# Autodesk Inventor assembly: Robot Assembly - 6 wheel - toughbox mini - 26x28 official version
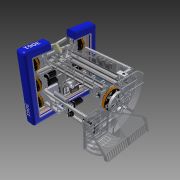
[picture p0: Inventor's stored thumbnail of the model, 180x180]
Saved by Autodesk Inventor 2013 (Build 170138000, 138)
## iProperties
Created: 2013-01-06
Part Number: Robot Assembly - 6 wheel - toughbox mini - 26x28 official version
Document SubType Name: Assembly
Designer: Moses
Mass: 49932.1 g
Surface Area: 138154 cm^2
Volume: 42618.2 cm^3
Density: 1.17161 g/cm^3
Author: Moses
## Documents named in this file (66)
- C:\Users\Arpan\Documents\GitHub\frc2013CAD\Robot Assembly - 6 wheel - toughbox mini - 26x28 official version.iam
- C:\Users\Arpan\Documents\GitHub\frc2013CAD\Drivetrain\Bearings\fr8zz-hex.ipt
- C:\Users\Arpan\Documents\GitHub\frc2013CAD\Drivetrain\Drive Wheel Assembly V2.iam
- C:\Users\Arpan\Documents\GitHub\frc2013CAD\Drivetrain\Standard Wheel Assembly V2.iam
- C:\Users\Arpan\Documents\GitHub\frc2013CAD\Drivetrain\Toughbox-mini\Toughbox-mini-hex-long.iam
- C:\Users\Arpan\Documents\GitHub\frc2013CAD\Drivetrain\6157K140 Shaft Collar\6157K140.ipt
- C:\Users\Arpan\Documents\GitHub\frc2013CAD\Drivetrain\Shaft Spacer Part1.ipt
- C:\Users\Arpan\Documents\GitHub\frc2013CAD\Drivetrain\Shaft Spacer Part2.ipt
- C:\Users\Arpan\Documents\GitHub\frc2013CAD\Drivetrain\Shaft Spacer Part3.ipt
- C:\Users\Arpan\Documents\GitHub\frc2013CAD\Drivetrain\Shaft Spacer Part4.ipt
- C:\Users\Arpan\Documents\GitHub\frc2013CAD\Drivetrain\Shaft Spacer Part5.ipt
- C:\Users\Arpan\Documents\GitHub\frc2013CAD\Drivetrain\Shaft Spacer Part6.ipt
- C:\Users\Arpan\Documents\GitHub\frc2013CAD\Drivetrain\6061K130 Shaft\6061K130.ipt
- C:\Users\Arpan\Documents\GitHub\frc2013CAD\Electrical\ELEC_CircuitBreaker_CB185-120.iam
- C:\Users\Arpan\Documents\GitHub\frc2013CAD\Electrical\CS_compactRIO_cRIO-FRC-II.ipt
- C:\Users\Arpan\Documents\GitHub\frc2013CAD\Electrical\CS_WirelessBridge_DAP1522.ipt
- C:\Users\Arpan\Documents\GitHub\frc2013CAD\Drivetrain\Pneumatic_Compressor_VIAIR_00090\Pneumatic_Compressor_VIAIR_00090.iam
- C:\Users\Arpan\Documents\GitHub\frc2013CAD\Drivetrain\Mounting Bracket V1.500 - (toughbox-mini - sheet metal).ipt
- C:\Users\Arpan\Documents\GitHub\frc2013CAD\Drivetrain\Mounting Bracket V1.500 - (toughbox-mini - sheet metal - underside).ipt
- C:\Users\Arpan\Documents\GitHub\frc2013CAD\Drivetrain\Bearing Block V1.500 Drivetrain.ipt
- C:\Users\Arpan\Documents\GitHub\frc2013CAD\Drivetrain\Shaft Mount V1.500 Drivetrain.ipt
- C:\Users\Arpan\Documents\GitHub\frc2013CAD\Launcher\Shooter\Shooter Assembly v2.iam
- C:\Users\Arpan\Documents\GitHub\frc2013CAD\Chassis\Chassis Assembly 26x28 Version\Chassis Assembly 26x28 Version.iam
- C:\Users\Arpan\Documents\GitHub\frc2013CAD\Chassis\Bumpers\Bumper Assembly1 (26x28 robot).iam
- C:\Users\Arpan\Documents\GitHub\frc2013CAD\Climber rough space budget version\arm assembly mount plate.ipt
- C:\Users\Arpan\Documents\GitHub\frc2013CAD\Cimber actual\main climber.iam
- C:\Users\Arpan\Documents\GitHub\frc2013CAD\Electrical\Mounting Board 3.ipt
- C:\Users\Arpan\Documents\GitHub\frc2013CAD\Drivetrain\Wheel Mount Support Plate - drive wheel.ipt
- C:\Users\Arpan\Documents\GitHub\frc2013CAD\Drivetrain\Wheel Mount Support Plate.ipt
- C:\Users\Arpan\Documents\GitHub\frc2013CAD\Chassis\Bumpers\Bumper Assembly2 (26x28 robot).iam
- C:\Users\Arpan\Documents\GitHub\frc2013CAD\Chassis\Bumpers\Bumper Assembly3 (26x28 robot).iam
- C:\Users\Arpan\Documents\GitHub\frc2013CAD\Chassis\Bumpers\Bumper Assembly4 (26x28 robot).iam
- C:\Users\Arpan\Documents\GitHub\frc2013CAD\Electrical\Electrical Board 1.iam
- C:\Users\Arpan\Documents\GitHub\frc2013CAD\Cimber actual\Arm Motor\arm bearing support.iam
- C:\Users\Arpan\Documents\GitHub\frc2013CAD\Cimber actual\Arm Motor\bracket for PG-71.ipt
- C:\Users\Arpan\Documents\GitHub\frc2013CAD\Cimber actual\Arm Motor\Imported Components\5972K322 bearing for motor\5972K322 bearing for motor.ipt
- C:\Users\Arpan\Documents\GitHub\frc2013CAD\Cimber actual\Arm Motor\Imported Components\PG-71-am-0914\PG-71-am-0914.ipt
- C:\Users\Arpan\Documents\GitHub\frc2013CAD\Cimber actual\Winch mount assenbly.iam
- C:\Users\Arpan\Documents\GitHub\frc2013CAD\Cimber actual\bearing 3 8 ths OD.ipt
- C:\Users\Arpan\Documents\GitHub\frc2013CAD\Cimber actual\14 inch shaft.ipt
- C:\Users\Arpan\Documents\GitHub\frc2013CAD\Cimber actual\winch support.ipt
- C:\Users\Arpan\Documents\GitHub\frc2013CAD\Cimber actual\anti - chain tension.ipt
- C:\Users\Arpan\Documents\GitHub\frc2013CAD\Cimber actual\spacer plate.ipt
- C:\Users\Arpan\Documents\GitHub\frc2013CAD\Cimber actual\V mount.ipt
- C:\Users\Arpan\Documents\GitHub\frc2013CAD\Cimber actual\nylon thing.ipt
- C:\Users\Arpan\Documents\GitHub\frc2013CAD\Cimber actual\p80 support post.iam
- C:\Users\Arpan\Documents\GitHub\frc2013CAD\Cimber actual\that thing mount.ipt
- C:\Users\Arpan\Documents\GitHub\frc2013CAD\Cimber actual\Hub for rachet.ipt
- C:\Users\Arpan\Documents\GitHub\frc2013CAD\Cimber actual\Part4.ipt
- C:\Users\Arpan\Documents\GitHub\frc2013CAD\Cimber actual\rachet gear analouge.ipt
- C:\Users\Arpan\Documents\GitHub\frc2013CAD\Cimber actual\cylinder.iam
- C:\Users\Arpan\Documents\GitHub\frc2013CAD\Cimber actual\tiny clevis.ipt
- C:\Users\Arpan\Documents\GitHub\frc2013CAD\Cimber actual\tube v.iam
- C:\Users\Arpan\Documents\GitHub\frc2013CAD\Cimber actual\paul mount.ipt
- C:\Users\Arpan\Documents\GitHub\frc2013CAD\Cimber actual\cylinder mount.ipt
- C:\Users\Arpan\Documents\GitHub\frc2013CAD\Cimber actual\passive hooks arpan style.iam.ipt
- C:\Users\Arpan\Documents\GitHub\frc2013CAD\Cimber actual\winch mount back support.ipt
- C:\Users\Arpan\Documents\GitHub\frc2013CAD\Cimber actual\ninja.ipt
- C:\Users\Arpan\Documents\GitHub\frc2013CAD\Climber rough space budget version\arm assembly mount plate 2.ipt
- C:\Users\Arpan\Documents\GitHub\frc2013CAD\Climber rough space budget version\arm assembly mount plate 3.ipt
- C:\Users\Arpan\Documents\GitHub\frc2013CAD\Cimber actual\P80 Mount Assembly V2.iam
- C:\Users\Arpan\Documents\GitHub\frc2013CAD\Cimber actual\Back Brace Mount V2.ipt
- C:\Users\Arpan\Documents\GitHub\frc2013CAD\Electrical\ELEC_Battery_NP18-12B.iam
- C:\Users\Arpan\Documents\GitHub\frc2013CAD\Pneumatics\Pneumatics_Clippard_AVT-32-16.iam
- C:\Users\Arpan\Documents\GitHub\frc2013CAD\Electrical\Circuit Breaker Mount.ipt
- passive hooks arpan style.iam
## Components (107 placed, 64 different names)
1. Chassis Assembly 26x28 Version:1 [sub-assembly] — Mate:1, Flush:1, Mate:2, Flush:4, Mate:3, Mate:4, Mate:5, Mate:8, Mate:9, Mate:10, Mate:17, Mate:18, Mate:19, Mate:20, Mate:21, Mate:26, Mate:27, Mate:28, Mate:29, Mate:34, Mate:35, Mate:36, Mate:37, Mate:42, Mate:43, Mate:44, Mate:47, Mate:48, Mate:51, Mate:52, Mate:55, Mate:83, Mate:84, Mate:85, Mate:89, Mate:98, Mate:99, Mate:100, Mate:101, Mate:115, Mate:116, Mate:117, Mate:118, Mate:119, Mate:120, Mate:125, Mate:126, Mate:127, Mate:128, Mate:129, Mate:130, Mate:132, Mate:136, Mate:153, Flush:17, Mate:154, Mate:155, Mate:159, Mate:190, Flush:162, Flush:191, Mate:194, Mate:195, Mate:196, Mate:197, Mate:198, Mate:199, Mate:200, Mate:201, Mate:202, Mate:203, Mate:204, Mate:205, Mate:206, Mate:207, Mate:208, Mate:209, Mate:210, Mate:211, Mate:212, Mate:213, Mate:214, Mate:215, Mate:216, Mate:217, Mate:218, Mate:219, Mate:220, Mate:221, Mate:222, Mate:223, Mate:249, Flush:193, Flush:194, Angle:4, Mate:255, Mate:256, Flush:196, Flush:197, Flush:204, Mate:271, Flush:206, Angle:5, Mate:278, Flush:208, Mate:279, Mate:282, Mate:284, Mate:286, Flush:213, Mate:288, Flush:214, Mate:289, Flush:216, Flush:222, Mate:310, Mate:311, Mate:312, Flush:233, Mate:316, Mate:317, Flush:235, Flush:237, Mate:319, Flush:238, Mate:321, Flush:239, Mate:323, Flush:215, Flush:217, Angle:11, Mate:328, Mate:329, Mate:330, Mate:331, Mate:332, Mate:333, Mate:334
2. Bumper Assembly1 (26x28 robot):1 [sub-assembly] — Mate:5, Mate:3, Flush:6, Flush:9, Flush:10
3. Bumper Assembly1 (26x28 robot):2 [sub-assembly] — Mate:1, Flush:1, Flush:3, Flush:2, Flush:7, Flush:8
4. Bumper Assembly2 (26x28 robot):1 [sub-assembly] — Mate:2, Flush:2, Flush:3, Flush:4, Mate:5, Flush:10
5. Bumper Assembly3 (26x28 robot):1 [sub-assembly] — Flush:9, Mate:5, Flush:6
6. Bumper Assembly4 (26x28 robot):1 [sub-assembly] — Mate:4, Flush:7, Flush:8
7. Wheel Mount Support Plate - drive wheel:1 — Mate:194, Mate:195, Mate:196
8. Wheel Mount Support Plate - drive wheel:2 — Mate:197, Mate:198, Mate:199
9. Wheel Mount Support Plate:1 — Mate:200, Mate:201, Mate:202
10. Wheel Mount Support Plate:2 — Mate:203, Mate:204, Mate:205
11. Wheel Mount Support Plate:3 — Mate:206, Mate:207, Mate:208
12. Wheel Mount Support Plate:4 — Mate:209, Mate:210, Mate:211
13. Wheel Mount Support Plate:5 — Mate:212, Mate:213, Mate:214
14. Wheel Mount Support Plate:6 — Mate:215, Mate:216, Mate:217
15. Wheel Mount Support Plate:7 — Mate:218, Mate:219, Mate:220
16. Wheel Mount Support Plate:8 — Mate:221, Mate:222, Mate:223
17. Pneumatic_Compressor_VIAIR_00090:1 [sub-assembly] — Mate:144, Mate:240, Mate:241, Mate:244, Mate:245
18. Shaft Spacer Part1:1 — Insert:111
19. Shaft Spacer Part2:1 — Insert:112
20. Shaft Spacer Part1:3 — Insert:113
21. Shaft Spacer Part2:2 — Insert:114
22. Shaft Spacer Part3:1 — Insert:115
23. Shaft Spacer Part3:2 — Insert:116
24. Shaft Spacer Part4:2 — Insert:117
25. Shaft Spacer Part4:1 — Insert:118
26. Shaft Spacer Part5:1 — Insert:119
27. Shaft Spacer Part5:2 — Insert:120
28. Shaft Spacer Part6:1 — Insert:121
29. Shaft Spacer Part6:2 — Insert:122
30. 6157K140:1 — Insert:107, Insert:113
31. 6157K140:2 — Insert:108, Insert:114
32. 6157K140:3 — Insert:110, Insert:111
33. 6157K140:4 — Insert:109, Insert:112
34. Toughbox-mini-hex-long:2 [sub-assembly] — Mate:131, Mate:132, Mate:133, Mate:134, Mate:135, Insert:118
35. Toughbox-mini-hex-long:1 [sub-assembly] — Mate:136, Mate:137, Mate:138, Mate:139, Mate:140, Insert:117
36. fr8zz-hex:1 — Insert:94, Insert:116
37. Bearing Block V1.500 Drivetrain:1 — Mate:83, Mate:84, Mate:85, Insert:106
38. Bearing Block V1.500 Drivetrain:2 — Mate:98, Mate:99, Mate:100, Insert:94
39. fr8zz-hex:2 — Insert:106, Insert:115
40. Mounting Bracket V1.500 - (toughbox-mini - sheet metal):1 — Mate:115, Mate:116, Mate:117, Mate:137, Mate:138
41. Mounting Bracket V1.500 - (toughbox-mini - sheet metal):2 — Mate:118, Mate:119, Mate:120, Mate:131, Mate:133
42. Mounting Bracket V1.500 - (toughbox-mini - sheet metal - underside):1 — Mate:125, Mate:126, Mate:127
43. Mounting Bracket V1.500 - (toughbox-mini - sheet metal - underside):2 — Mate:128, Mate:129, Mate:130
44. Shaft Mount V1.500 Drivetrain:8 — Mate:34, Mate:35, Mate:51, Insert:121
45. Shaft Mount V1.500 Drivetrain:7 — Mate:28, Mate:29, Mate:48, Insert:110
46. Shaft Mount V1.500 Drivetrain:6 — Mate:42, Mate:43, Mate:47, Insert:122
47. Shaft Mount V1.500 Drivetrain:5 — Mate:36, Mate:37, Mate:44, Insert:107
48. Shaft Mount V1.500 Drivetrain:4 — Mate:26, Mate:27, Mate:55, Insert:7, Insert:109
49. Shaft Mount V1.500 Drivetrain:3 — Mate:20, Mate:21, Mate:52, Insert:5, Insert:119
50. Shaft Mount V1.500 Drivetrain:2 — Mate:17, Mate:18, Mate:19, Insert:2, Insert:108
51. Shaft Mount V1.500 Drivetrain:1 — Mate:8, Mate:9, Mate:10, Insert:1, Insert:120
52. 6061K130:4 — Insert:7, Mate:21
53. 6061K130:3 — Insert:5, Mate:22
54. 6061K130:2 — Insert:2, Mate:19
55. 6061K130:1 — Insert:1, Mate:17
56. Standard Wheel Assembly V2:3 [sub-assembly] — Mate:17, Flush:13, Rotation:1
57. Drive Wheel Assembly V2:1 [sub-assembly] — Mate:89, Flush:13, Flush:15, Mate:139, Mate:140, Rotation:1, Rotation:2, Tangent:3
58. Standard Wheel Assembly V2:1 [sub-assembly] — Mate:19, Flush:15, Rotation:2
59. Standard Wheel Assembly V2:2 [sub-assembly] — Mate:21, Flush:11, Rotation:4
60. Standard Wheel Assembly V2:4 [sub-assembly] — Mate:22, Flush:12, Rotation:3
61. Drive Wheel Assembly V2:2 [sub-assembly] — Mate:101, Flush:11, Flush:12, Mate:134, Mate:135, Rotation:3, Rotation:4
62. Circuit Breaker Mount:1 — Mate:335, Mate:246, Mate:338, Mate:13, Mate:339, Mate:340
63. Pneumatics_Clippard_AVT-32-16:1 [sub-assembly] — Tangent:4, Angle:12, Mate:334, Tangent:5
64. ELEC_Battery_NP18-12B:1 [sub-assembly] — Mate:331, Mate:332, Mate:333
65. Mounting Board 3:1 — Mate:190, Flush:162, Mate:16, Mate:188, Mate:189, Flush:191, Mate:144, Mate:240, Mate:241, Mate:244, Mate:245
66. Electrical Board 1:1 [sub-assembly] — Mate:242, Mate:243, Flush:192
67. CS_WirelessBridge_DAP1522:1 — Flush:152, Mate:164, Flush:224
68. CS_compactRIO_cRIO-FRC-II:1 — Mate:16, Mate:188, Mate:189
69. ELEC_CircuitBreaker_CB185-120:1 [sub-assembly] — Mate:246, Mate:338, Mate:13
70. Shooter Assembly v2:1 [sub-assembly] — Mate:153, Flush:17, Mate:154, Mate:159, Mate:164, Flush:152, Flush:224, Mate:242, Mate:243, Flush:192, Mate:258, Mate:285, Flush:211, Mate:326, Flush:240, Tangent:4, Angle:12, Tangent:5
71. main climber:1 [sub-assembly] — Tangent:2, Mate:282, Mate:308, Mate:309, Mate:318, Mate:320, Mate:322, Angle:11
72. arm bearing support:1 [sub-assembly] — Mate:249, Flush:193, Mate:252, Flush:195
73. bracket for PG-71:1 — Flush:194, Mate:253, Mate:323, Mate:324
74. arm assembly mount plate:2 — Mate:155, Mate:318, Flush:237, Mate:328, Mate:329
75. 5972K322 bearing for motor:1 — Mate:252, Flush:195, Mate:254, Mate:325
76. PG-71-am-0914:1 — Mate:253, Mate:254, Mate:324, Mate:325
77. Back Brace Mount V2:1 — Mate:326, Flush:240, Mate:327, Mate:335, Mate:339, Mate:340
78. Winch mount assenbly:1 [sub-assembly] — Mate:255, Flush:197, Mate:257, Mate:258, Mate:259, Mate:262, Mate:269, Mate:270, Flush:205, Flush:234
79. bearing 3 8 ths OD:1 — Mate:259, Mate:262, Mate:263
80. Winch mount assenbly:2 [sub-assembly] — Mate:256, Flush:196, Mate:257, Mate:260, Mate:261, Flush:207, Mate:300, Flush:227, Mate:301, Mate:302, Mate:304, Mate:305, Mate:314, Mate:315
81. bearing 3 8 ths OD:2 — Mate:260, Mate:261
82. 14 inch shaft:1 — Mate:263, Mate:290, Mate:292
83. winch support:2 — Flush:204, Mate:269, Mate:270, Flush:205, Mate:272, Mate:273, Mate:274
84. winch support:3 — Mate:271, Flush:206, Flush:207
85. anti - chain tension:1 — Mate:272, Mate:273, Mate:274, Mate:276, Mate:277
86. spacer plate:1 — Mate:276, Mate:277
87. V mount:1 — Mate:278, Flush:208, Mate:279, Mate:283, Flush:210, Flush:215, Flush:217, Mate:298, Mate:299
88. nylon thing:1 — Mate:283, Mate:284, Flush:210
89. P80 Mount Assembly V2:1 [sub-assembly] — Mate:285, Flush:211, Mate:287, Mate:327
90. that thing mount:1 — Mate:288, Flush:214, Angle:10
91. that thing mount:2 — Mate:289, Flush:216
92. p80 support post:1 [sub-assembly] — Mate:286, Mate:287, Flush:213, Flush:236
93. Hub for rachet:1 — Mate:290, Mate:293
94. Part4:1
95. rachet gear analouge:1 — Mate:292, Mate:293
96. cylinder:1 [sub-assembly] — Mate:306, Angle:6, Flush:229, Mate:307, Flush:230, Flush:231
97. tube v:1 [sub-assembly] — Mate:298, Mate:299, Flush:222
98. paul mount:1 — Mate:300, Flush:227, Mate:301, Flush:228
99. cylinder mount:2 — Mate:304, Flush:228, Mate:305, Angle:7, Mate:307, Flush:230, Flush:231, Mate:302
100. tiny clevis:1 — Mate:306, Angle:6, Angle:7, Flush:229
101. passive hooks arpan style.iam:1 — Mate:308, Mate:311, Angle:9, Angle:10
102. passive hooks arpan style.iam:2 — Mate:309, Mate:310, Angle:9
103. winch mount back support:1 — Mate:312, Flush:233, Flush:234
104. ninja:1 — Mate:317, Flush:235, Flush:236
105. winch mount back support:2 — Mate:314, Mate:315, Mate:316
106. arm assembly mount plate 2:1 — Mate:319, Flush:238, Mate:320, Mate:330
107. arm assembly mount plate 3:1 — Mate:321, Mate:322, Flush:239
## Relationships (273: Mate 185, Flush 50, Insert 22, Angle 8, RelateRotation 4, Tangent 4)
- Mate:1: Chassis Assembly 26x28 Version:1 ↔ Bumper Assembly1 (26x28 robot):2
- Flush:1: Chassis Assembly 26x28 Version:1 ↔ Bumper Assembly1 (26x28 robot):2
- Mate:2: Chassis Assembly 26x28 Version:1 ↔ Bumper Assembly2 (26x28 robot):1
- Flush:2: Bumper Assembly1 (26x28 robot):2 ↔ Bumper Assembly2 (26x28 robot):1
- Flush:3: Bumper Assembly1 (26x28 robot):2 ↔ Bumper Assembly2 (26x28 robot):1
- Flush:4 (-69.85 mm): Chassis Assembly 26x28 Version:1 ↔ Bumper Assembly2 (26x28 robot):1
- Mate:5: Bumper Assembly1 (26x28 robot):1 ↔ Bumper Assembly2 (26x28 robot):1
- Mate:3: Chassis Assembly 26x28 Version:1 ↔ Bumper Assembly1 (26x28 robot):1
- Flush:6: Bumper Assembly1 (26x28 robot):1 ↔ Bumper Assembly3 (26x28 robot):1
- Mate:4: Chassis Assembly 26x28 Version:1 ↔ Bumper Assembly4 (26x28 robot):1
- Flush:7: Bumper Assembly1 (26x28 robot):2 ↔ Bumper Assembly4 (26x28 robot):1
- Flush:8: Bumper Assembly1 (26x28 robot):2 ↔ Bumper Assembly4 (26x28 robot):1
- Flush:9: Bumper Assembly1 (26x28 robot):1 ↔ Bumper Assembly3 (26x28 robot):1
- Flush:10: Bumper Assembly1 (26x28 robot):1 ↔ Bumper Assembly2 (26x28 robot):1
- Mate:5: Chassis Assembly 26x28 Version:1 ↔ Bumper Assembly3 (26x28 robot):1
- Insert:1 (-6.35 mm): Shaft Mount V1.500 Drivetrain:1 ↔ 6061K130:1
- Insert:2 (-6.35 mm): Shaft Mount V1.500 Drivetrain:2 ↔ 6061K130:2
- Insert:5 (-6.35 mm): Shaft Mount V1.500 Drivetrain:3 ↔ 6061K130:3
- Insert:7 (-6.35 mm): Shaft Mount V1.500 Drivetrain:4 ↔ 6061K130:4
- Mate:8: Chassis Assembly 26x28 Version:1 ↔ Shaft Mount V1.500 Drivetrain:1
- Mate:9: Chassis Assembly 26x28 Version:1 ↔ Shaft Mount V1.500 Drivetrain:1
- Mate:10: Chassis Assembly 26x28 Version:1 ↔ Shaft Mount V1.500 Drivetrain:1
- Mate:17: Chassis Assembly 26x28 Version:1 ↔ Shaft Mount V1.500 Drivetrain:2
- Mate:18: Chassis Assembly 26x28 Version:1 ↔ Shaft Mount V1.500 Drivetrain:2
- Mate:19: Chassis Assembly 26x28 Version:1 ↔ Shaft Mount V1.500 Drivetrain:2
- Mate:20: Chassis Assembly 26x28 Version:1 ↔ Shaft Mount V1.500 Drivetrain:3
- Mate:21: Chassis Assembly 26x28 Version:1 ↔ Shaft Mount V1.500 Drivetrain:3
- Mate:26: Chassis Assembly 26x28 Version:1 ↔ Shaft Mount V1.500 Drivetrain:4
- Mate:27: Chassis Assembly 26x28 Version:1 ↔ Shaft Mount V1.500 Drivetrain:4
- Mate:28: Chassis Assembly 26x28 Version:1 ↔ Shaft Mount V1.500 Drivetrain:7
- Mate:29: Chassis Assembly 26x28 Version:1 ↔ Shaft Mount V1.500 Drivetrain:7
- Mate:34: Chassis Assembly 26x28 Version:1 ↔ Shaft Mount V1.500 Drivetrain:8
- Mate:35: Chassis Assembly 26x28 Version:1 ↔ Shaft Mount V1.500 Drivetrain:8
- Mate:36: Chassis Assembly 26x28 Version:1 ↔ Shaft Mount V1.500 Drivetrain:5
- Mate:37: Chassis Assembly 26x28 Version:1 ↔ Shaft Mount V1.500 Drivetrain:5
- Mate:42: Chassis Assembly 26x28 Version:1 ↔ Shaft Mount V1.500 Drivetrain:6
- Mate:43: Chassis Assembly 26x28 Version:1 ↔ Shaft Mount V1.500 Drivetrain:6
- Mate:44: Chassis Assembly 26x28 Version:1 ↔ Shaft Mount V1.500 Drivetrain:5
- Mate:47: Chassis Assembly 26x28 Version:1 ↔ Shaft Mount V1.500 Drivetrain:6
- Mate:48: Chassis Assembly 26x28 Version:1 ↔ Shaft Mount V1.500 Drivetrain:7
- Mate:51: Chassis Assembly 26x28 Version:1 ↔ Shaft Mount V1.500 Drivetrain:8
- Mate:52: Chassis Assembly 26x28 Version:1 ↔ Shaft Mount V1.500 Drivetrain:3
- Mate:55: Chassis Assembly 26x28 Version:1 ↔ Shaft Mount V1.500 Drivetrain:4
- Mate:17: 6061K130:1 ↔ Standard Wheel Assembly V2:3
- Mate:19: 6061K130:2 ↔ Standard Wheel Assembly V2:1
- Mate:21: 6061K130:4 ↔ Standard Wheel Assembly V2:2
- Mate:22: 6061K130:3 ↔ Standard Wheel Assembly V2:4
- Mate:83: Chassis Assembly 26x28 Version:1 ↔ Bearing Block V1.500 Drivetrain:1
- Mate:84: Chassis Assembly 26x28 Version:1 ↔ Bearing Block V1.500 Drivetrain:1
- Mate:85: Chassis Assembly 26x28 Version:1 ↔ Bearing Block V1.500 Drivetrain:1
- Mate:89 (6.35 mm): Chassis Assembly 26x28 Version:1 ↔ Drive Wheel Assembly V2:1
- Insert:94: fr8zz-hex:1 ↔ Bearing Block V1.500 Drivetrain:2
- Mate:98: Chassis Assembly 26x28 Version:1 ↔ Bearing Block V1.500 Drivetrain:2
- Mate:99: Chassis Assembly 26x28 Version:1 ↔ Bearing Block V1.500 Drivetrain:2
- Mate:100: Chassis Assembly 26x28 Version:1 ↔ Bearing Block V1.500 Drivetrain:2
- Mate:101 (6.35 mm): Chassis Assembly 26x28 Version:1 ↔ Drive Wheel Assembly V2:2
- Insert:106: Bearing Block V1.500 Drivetrain:1 ↔ fr8zz-hex:2
- Mate:115: Chassis Assembly 26x28 Version:1 ↔ Mounting Bracket V1.500 - (toughbox-mini - sheet metal):1
- Mate:116: Chassis Assembly 26x28 Version:1 ↔ Mounting Bracket V1.500 - (toughbox-mini - sheet metal):1
- Mate:117: Chassis Assembly 26x28 Version:1 ↔ Mounting Bracket V1.500 - (toughbox-mini - sheet metal):1
- Mate:118: Chassis Assembly 26x28 Version:1 ↔ Mounting Bracket V1.500 - (toughbox-mini - sheet metal):2
- Mate:119: Chassis Assembly 26x28 Version:1 ↔ Mounting Bracket V1.500 - (toughbox-mini - sheet metal):2
- Mate:120: Chassis Assembly 26x28 Version:1 ↔ Mounting Bracket V1.500 - (toughbox-mini - sheet metal):2
- Flush:11: Standard Wheel Assembly V2:2 ↔ Drive Wheel Assembly V2:2
- Flush:12: Standard Wheel Assembly V2:4 ↔ Drive Wheel Assembly V2:2
- Flush:13: Standard Wheel Assembly V2:3 ↔ Drive Wheel Assembly V2:1
- Mate:125: Chassis Assembly 26x28 Version:1 ↔ Mounting Bracket V1.500 - (toughbox-mini - sheet metal - underside):1
- Mate:126: Chassis Assembly 26x28 Version:1 ↔ Mounting Bracket V1.500 - (toughbox-mini - sheet metal - underside):1
- Mate:127: Chassis Assembly 26x28 Version:1 ↔ Mounting Bracket V1.500 - (toughbox-mini - sheet metal - underside):1
- Mate:128: Chassis Assembly 26x28 Version:1 ↔ Mounting Bracket V1.500 - (toughbox-mini - sheet metal - underside):2
- Mate:129: Chassis Assembly 26x28 Version:1 ↔ Mounting Bracket V1.500 - (toughbox-mini - sheet metal - underside):2
- Mate:130: Chassis Assembly 26x28 Version:1 ↔ Mounting Bracket V1.500 - (toughbox-mini - sheet metal - underside):2
- Flush:15: Drive Wheel Assembly V2:1 ↔ Standard Wheel Assembly V2:1
- Mate:131: Toughbox-mini-hex-long:2 ↔ Mounting Bracket V1.500 - (toughbox-mini - sheet metal):2
- Mate:132: Chassis Assembly 26x28 Version:1 ↔ Toughbox-mini-hex-long:2
- Mate:133: Toughbox-mini-hex-long:2 ↔ Mounting Bracket V1.500 - (toughbox-mini - sheet metal):2
- Mate:134: Toughbox-mini-hex-long:2 ↔ Drive Wheel Assembly V2:2
- Mate:135: Toughbox-mini-hex-long:2 ↔ Drive Wheel Assembly V2:2
- Mate:136: Chassis Assembly 26x28 Version:1 ↔ Toughbox-mini-hex-long:1
- Mate:137: Toughbox-mini-hex-long:1 ↔ Mounting Bracket V1.500 - (toughbox-mini - sheet metal):1
- Mate:138: Toughbox-mini-hex-long:1 ↔ Mounting Bracket V1.500 - (toughbox-mini - sheet metal):1
- Mate:139: Toughbox-mini-hex-long:1 ↔ Drive Wheel Assembly V2:1
- Mate:140: Toughbox-mini-hex-long:1 ↔ Drive Wheel Assembly V2:1
- Rotation:1 [RelateRotation] (1 ul): Standard Wheel Assembly V2:3 ↔ Drive Wheel Assembly V2:1
- Rotation:2 [RelateRotation] (1 ul): Drive Wheel Assembly V2:1 ↔ Standard Wheel Assembly V2:1
- Rotation:3 [RelateRotation] (1 ul): Standard Wheel Assembly V2:4 ↔ Drive Wheel Assembly V2:2
- Rotation:4 [RelateRotation] (1 ul): Standard Wheel Assembly V2:2 ↔ Drive Wheel Assembly V2:2
- Insert:107: 6157K140:1 ↔ Shaft Mount V1.500 Drivetrain:5
- Insert:108: 6157K140:2 ↔ Shaft Mount V1.500 Drivetrain:2
- Insert:109: 6157K140:4 ↔ Shaft Mount V1.500 Drivetrain:4
- Insert:110: 6157K140:3 ↔ Shaft Mount V1.500 Drivetrain:7
- Insert:111: Shaft Spacer Part1:1 ↔ 6157K140:3
- Insert:112: Shaft Spacer Part2:1 ↔ 6157K140:4
- Insert:113: Shaft Spacer Part1:3 ↔ 6157K140:1
- Insert:114: Shaft Spacer Part2:2 ↔ 6157K140:2
- Insert:115: Shaft Spacer Part3:1 ↔ fr8zz-hex:2
- Insert:116: Shaft Spacer Part3:2 ↔ fr8zz-hex:1
- Insert:117: Shaft Spacer Part4:2 ↔ Toughbox-mini-hex-long:1
- Insert:118: Shaft Spacer Part4:1 ↔ Toughbox-mini-hex-long:2
- Insert:119: Shaft Spacer Part5:1 ↔ Shaft Mount V1.500 Drivetrain:3
- Insert:120: Shaft Spacer Part5:2 ↔ Shaft Mount V1.500 Drivetrain:1
- Insert:121: Shaft Spacer Part6:1 ↔ Shaft Mount V1.500 Drivetrain:8
- Insert:122: Shaft Spacer Part6:2 ↔ Shaft Mount V1.500 Drivetrain:6
- Mate:16: Mounting Board 3:1 ↔ CS_compactRIO_cRIO-FRC-II:1
- Mate:144: Pneumatic_Compressor_VIAIR_00090:1 ↔ Mounting Board 3:1
- Flush:152: CS_WirelessBridge_DAP1522:1 ↔ Shooter Assembly v2:1
- Mate:153: Chassis Assembly 26x28 Version:1 ↔ Shooter Assembly v2:1
- Flush:17: Chassis Assembly 26x28 Version:1 ↔ Shooter Assembly v2:1
- Mate:154: Chassis Assembly 26x28 Version:1 ↔ Shooter Assembly v2:1
- Mate:155: Chassis Assembly 26x28 Version:1 ↔ arm assembly mount plate:2
- Mate:159: Chassis Assembly 26x28 Version:1 ↔ Shooter Assembly v2:1
- Mate:164: CS_WirelessBridge_DAP1522:1 ↔ Shooter Assembly v2:1
- Mate:188: Mounting Board 3:1 ↔ CS_compactRIO_cRIO-FRC-II:1
- Mate:189: Mounting Board 3:1 ↔ CS_compactRIO_cRIO-FRC-II:1
- Mate:190: Chassis Assembly 26x28 Version:1 ↔ Mounting Board 3:1
- Flush:162: Chassis Assembly 26x28 Version:1 ↔ Mounting Board 3:1
- Flush:191: Chassis Assembly 26x28 Version:1 ↔ Mounting Board 3:1
- Mate:194: Chassis Assembly 26x28 Version:1 ↔ Wheel Mount Support Plate - drive wheel:1
- Mate:195: Chassis Assembly 26x28 Version:1 ↔ Wheel Mount Support Plate - drive wheel:1
- Mate:196: Chassis Assembly 26x28 Version:1 ↔ Wheel Mount Support Plate - drive wheel:1
- Mate:197: Chassis Assembly 26x28 Version:1 ↔ Wheel Mount Support Plate - drive wheel:2
- Mate:198: Chassis Assembly 26x28 Version:1 ↔ Wheel Mount Support Plate - drive wheel:2
- Mate:199: Chassis Assembly 26x28 Version:1 ↔ Wheel Mount Support Plate - drive wheel:2
- Mate:200: Chassis Assembly 26x28 Version:1 ↔ Wheel Mount Support Plate:1
- Mate:201: Chassis Assembly 26x28 Version:1 ↔ Wheel Mount Support Plate:1
- Mate:202: Chassis Assembly 26x28 Version:1 ↔ Wheel Mount Support Plate:1
- Mate:203: Chassis Assembly 26x28 Version:1 ↔ Wheel Mount Support Plate:2
- Mate:204: Chassis Assembly 26x28 Version:1 ↔ Wheel Mount Support Plate:2
- Mate:205: Chassis Assembly 26x28 Version:1 ↔ Wheel Mount Support Plate:2
- Mate:206: Chassis Assembly 26x28 Version:1 ↔ Wheel Mount Support Plate:3
- Mate:207: Chassis Assembly 26x28 Version:1 ↔ Wheel Mount Support Plate:3
- Mate:208: Chassis Assembly 26x28 Version:1 ↔ Wheel Mount Support Plate:3
- Mate:209: Chassis Assembly 26x28 Version:1 ↔ Wheel Mount Support Plate:4
- Mate:210: Chassis Assembly 26x28 Version:1 ↔ Wheel Mount Support Plate:4
- Mate:211: Chassis Assembly 26x28 Version:1 ↔ Wheel Mount Support Plate:4
- Mate:212: Chassis Assembly 26x28 Version:1 ↔ Wheel Mount Support Plate:5
- Mate:213: Chassis Assembly 26x28 Version:1 ↔ Wheel Mount Support Plate:5
- Mate:214: Chassis Assembly 26x28 Version:1 ↔ Wheel Mount Support Plate:5
- Mate:215: Chassis Assembly 26x28 Version:1 ↔ Wheel Mount Support Plate:6
- Mate:216: Chassis Assembly 26x28 Version:1 ↔ Wheel Mount Support Plate:6
- Mate:217: Chassis Assembly 26x28 Version:1 ↔ Wheel Mount Support Plate:6
- Mate:218: Chassis Assembly 26x28 Version:1 ↔ Wheel Mount Support Plate:7
- Mate:219: Chassis Assembly 26x28 Version:1 ↔ Wheel Mount Support Plate:7
- Mate:220: Chassis Assembly 26x28 Version:1 ↔ Wheel Mount Support Plate:7
- Mate:221: Chassis Assembly 26x28 Version:1 ↔ Wheel Mount Support Plate:8
- Mate:222: Chassis Assembly 26x28 Version:1 ↔ Wheel Mount Support Plate:8
- Mate:223: Chassis Assembly 26x28 Version:1 ↔ Wheel Mount Support Plate:8
- Flush:224: CS_WirelessBridge_DAP1522:1 ↔ Shooter Assembly v2:1
- Mate:240: Pneumatic_Compressor_VIAIR_00090:1 ↔ Mounting Board 3:1
- Mate:241: Pneumatic_Compressor_VIAIR_00090:1 ↔ Mounting Board 3:1
- Mate:242 (12.7 mm): Electrical Board 1:1 ↔ Shooter Assembly v2:1
- Mate:243: Electrical Board 1:1 ↔ Shooter Assembly v2:1
- Flush:192: Electrical Board 1:1 ↔ Shooter Assembly v2:1
- Mate:244: Pneumatic_Compressor_VIAIR_00090:1 ↔ Mounting Board 3:1
- Mate:245: Pneumatic_Compressor_VIAIR_00090:1 ↔ Mounting Board 3:1
- Mate:246: Circuit Breaker Mount:1 ↔ ELEC_CircuitBreaker_CB185-120:1
- Mate:249: Chassis Assembly 26x28 Version:1 ↔ arm bearing support:1
- Flush:193 (-3.175 mm): Chassis Assembly 26x28 Version:1 ↔ arm bearing support:1
- Flush:194: Chassis Assembly 26x28 Version:1 ↔ bracket for PG-71:1
- Angle:4 (0 deg): Chassis Assembly 26x28 Version:1
- Tangent:2: main climber:1
- Mate:252: arm bearing support:1 ↔ 5972K322 bearing for motor:1
- Flush:195: arm bearing support:1 ↔ 5972K322 bearing for motor:1
- Mate:253: bracket for PG-71:1 ↔ PG-71-am-0914:1
- Mate:254: 5972K322 bearing for motor:1 ↔ PG-71-am-0914:1
- Mate:255: Chassis Assembly 26x28 Version:1 ↔ Winch mount assenbly:1
- Mate:256: Chassis Assembly 26x28 Version:1 ↔ Winch mount assenbly:2
- Flush:196: Chassis Assembly 26x28 Version:1 ↔ Winch mount assenbly:2
- Flush:197: Chassis Assembly 26x28 Version:1 ↔ Winch mount assenbly:1
- Mate:257: Winch mount assenbly:1 ↔ Winch mount assenbly:2
- Mate:258: Shooter Assembly v2:1 ↔ Winch mount assenbly:1
- Mate:259: Winch mount assenbly:1 ↔ bearing 3 8 ths OD:1
- Mate:260: Winch mount assenbly:2 ↔ bearing 3 8 ths OD:2
- Mate:261: Winch mount assenbly:2 ↔ bearing 3 8 ths OD:2
- Mate:262: Winch mount assenbly:1 ↔ bearing 3 8 ths OD:1
- Mate:263: bearing 3 8 ths OD:1 ↔ 14 inch shaft:1
- Flush:204: Chassis Assembly 26x28 Version:1 ↔ winch support:2
- Mate:269: Winch mount assenbly:1 ↔ winch support:2
- Mate:270: Winch mount assenbly:1 ↔ winch support:2
- Flush:205: Winch mount assenbly:1 ↔ winch support:2
- Mate:271: Chassis Assembly 26x28 Version:1 ↔ winch support:3
- Flush:206: Chassis Assembly 26x28 Version:1 ↔ winch support:3
- Flush:207: Winch mount assenbly:2 ↔ winch support:3
- Mate:272: winch support:2 ↔ anti - chain tension:1
- Mate:273: winch support:2 ↔ anti - chain tension:1
- Mate:274: winch support:2 ↔ anti - chain tension:1
- Mate:276: anti - chain tension:1 ↔ spacer plate:1
- Mate:277: anti - chain tension:1 ↔ spacer plate:1
- Angle:5 (0 deg): Chassis Assembly 26x28 Version:1
- Tangent:3: Drive Wheel Assembly V2:1
- Mate:278: Chassis Assembly 26x28 Version:1 ↔ V mount:1
- Flush:208: Chassis Assembly 26x28 Version:1 ↔ V mount:1
- Mate:279 (139.7 mm): Chassis Assembly 26x28 Version:1 ↔ V mount:1
- Mate:282 (7.7089 mm): Chassis Assembly 26x28 Version:1 ↔ main climber:1
- Mate:283: V mount:1 ↔ nylon thing:1
- Mate:284 (12.7 mm): Chassis Assembly 26x28 Version:1 ↔ nylon thing:1
- Flush:210: V mount:1 ↔ nylon thing:1
- Mate:285: Shooter Assembly v2:1 ↔ P80 Mount Assembly V2:1
- Flush:211: Shooter Assembly v2:1 ↔ P80 Mount Assembly V2:1
- Mate:286: Chassis Assembly 26x28 Version:1 ↔ p80 support post:1
- Mate:287: P80 Mount Assembly V2:1 ↔ p80 support post:1
- Flush:213: Chassis Assembly 26x28 Version:1 ↔ p80 support post:1
- Mate:288: Chassis Assembly 26x28 Version:1 ↔ that thing mount:1
- Flush:214: Chassis Assembly 26x28 Version:1 ↔ that thing mount:1
- Flush:215 (165.1 mm): Chassis Assembly 26x28 Version:1 ↔ V mount:1
- Mate:289: Chassis Assembly 26x28 Version:1 ↔ that thing mount:2
- Flush:216: Chassis Assembly 26x28 Version:1 ↔ that thing mount:2
- Flush:217 (165.1 mm): Chassis Assembly 26x28 Version:1 ↔ V mount:1
- Mate:290: 14 inch shaft:1 ↔ Hub for rachet:1
- Mate:292: 14 inch shaft:1 ↔ rachet gear analouge:1
- Mate:293: Hub for rachet:1 ↔ rachet gear analouge:1
- Mate:298: V mount:1 ↔ tube v:1
- Mate:299: V mount:1 ↔ tube v:1
- Flush:222: Chassis Assembly 26x28 Version:1 ↔ tube v:1
- Mate:300: Winch mount assenbly:2 ↔ paul mount:1
- Flush:227: Winch mount assenbly:2 ↔ paul mount:1
- Mate:301: Winch mount assenbly:2 ↔ paul mount:1
- Mate:302: Winch mount assenbly:2 ↔ cylinder mount:2
- Mate:304: Winch mount assenbly:2 ↔ cylinder mount:2
- Flush:228: paul mount:1 ↔ cylinder mount:2
- Mate:305: Winch mount assenbly:2 ↔ cylinder mount:2
- Mate:306: cylinder:1 ↔ tiny clevis:1
- Angle:6 (180 deg): cylinder:1 ↔ tiny clevis:1
- Angle:7 (180 deg): cylinder mount:2 ↔ tiny clevis:1
- Flush:229: cylinder:1 ↔ tiny clevis:1
- Mate:307: cylinder:1 ↔ cylinder mount:2
- Flush:230 (38.1 mm): cylinder:1 ↔ cylinder mount:2
- Flush:231 (12.7 mm): cylinder:1 ↔ cylinder mount:2
- Mate:308: main climber:1 ↔ passive hooks arpan style.iam:1
- Mate:309: main climber:1 ↔ passive hooks arpan style.iam:2
- Mate:310 (3.175 mm): Chassis Assembly 26x28 Version:1 ↔ passive hooks arpan style.iam:2
- Mate:311 (3.175 mm): Chassis Assembly 26x28 Version:1 ↔ passive hooks arpan style.iam:1
- Angle:9 (0 deg): passive hooks arpan style.iam:1 ↔ passive hooks arpan style.iam:2
- Angle:10 (50 deg): that thing mount:1 ↔ passive hooks arpan style.iam:1
- Mate:312: Chassis Assembly 26x28 Version:1 ↔ winch mount back support:1
- Flush:233: Chassis Assembly 26x28 Version:1 ↔ winch mount back support:1
- Flush:234: Winch mount assenbly:1 ↔ winch mount back support:1
- Mate:314: Winch mount assenbly:2 ↔ winch mount back support:2
- Mate:315: Winch mount assenbly:2 ↔ winch mount back support:2
- Mate:316: Chassis Assembly 26x28 Version:1 ↔ winch mount back support:2
- Mate:317: Chassis Assembly 26x28 Version:1 ↔ ninja:1
- Flush:235: Chassis Assembly 26x28 Version:1 ↔ ninja:1
- Flush:236: p80 support post:1 ↔ ninja:1
- Mate:318: main climber:1 ↔ arm assembly mount plate:2
- Flush:237: Chassis Assembly 26x28 Version:1 ↔ arm assembly mount plate:2
- Mate:319: Chassis Assembly 26x28 Version:1 ↔ arm assembly mount plate 2:1
- Flush:238: Chassis Assembly 26x28 Version:1 ↔ arm assembly mount plate 2:1
- Mate:320: main climber:1 ↔ arm assembly mount plate 2:1
- Mate:321: Chassis Assembly 26x28 Version:1 ↔ arm assembly mount plate 3:1
- Mate:322: main climber:1 ↔ arm assembly mount plate 3:1
- Flush:239: Chassis Assembly 26x28 Version:1 ↔ arm assembly mount plate 3:1
- Mate:323: Chassis Assembly 26x28 Version:1 ↔ bracket for PG-71:1
- Mate:324: bracket for PG-71:1 ↔ PG-71-am-0914:1
- Mate:325: 5972K322 bearing for motor:1 ↔ PG-71-am-0914:1
- Mate:326: Shooter Assembly v2:1 ↔ Back Brace Mount V2:1
- Flush:240: Shooter Assembly v2:1 ↔ Back Brace Mount V2:1
- Mate:327: Back Brace Mount V2:1 ↔ P80 Mount Assembly V2:1
- Angle:11 (90 deg): Chassis Assembly 26x28 Version:1 ↔ main climber:1
- Mate:328: Chassis Assembly 26x28 Version:1 ↔ arm assembly mount plate:2
- Mate:329: Chassis Assembly 26x28 Version:1 ↔ arm assembly mount plate:2
- Mate:330: Chassis Assembly 26x28 Version:1 ↔ arm assembly mount plate 2:1
- Mate:331: Chassis Assembly 26x28 Version:1 ↔ ELEC_Battery_NP18-12B:1
- Mate:332: Chassis Assembly 26x28 Version:1 ↔ ELEC_Battery_NP18-12B:1
- Mate:333: Chassis Assembly 26x28 Version:1 ↔ ELEC_Battery_NP18-12B:1
- Tangent:4: Pneumatics_Clippard_AVT-32-16:1 ↔ Shooter Assembly v2:1
- Angle:12 (0 deg): Pneumatics_Clippard_AVT-32-16:1 ↔ Shooter Assembly v2:1
- Mate:334 (152.4 mm): Chassis Assembly 26x28 Version:1 ↔ Pneumatics_Clippard_AVT-32-16:1
- Tangent:5: Pneumatics_Clippard_AVT-32-16:1 ↔ Shooter Assembly v2:1
- Mate:335: Circuit Breaker Mount:1 ↔ Back Brace Mount V2:1
- Mate:338: Circuit Breaker Mount:1 ↔ ELEC_CircuitBreaker_CB185-120:1
- Mate:13: Circuit Breaker Mount:1 ↔ ELEC_CircuitBreaker_CB185-120:1
- Mate:339: Circuit Breaker Mount:1 ↔ Back Brace Mount V2:1
- Mate:340: Circuit Breaker Mount:1 ↔ Back Brace Mount V2:1
